# Autodesk Inventor assembly: staticFrame
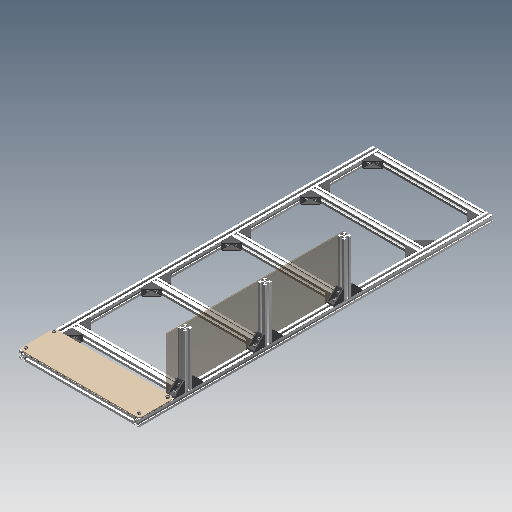
[picture p0: Inventor's stored thumbnail of the model, 512x512]
Saved by Autodesk Inventor 2018 (Build 220112000, 112)
## iProperties
Created: 2017-04-19
Part Number: staticFrame
Document SubType Name: Assembly
Designer: sawaiz
Author: sawaiz
## Documents named in this file (7)
- C:\Users\sawaiz\OneDrive\projects\sPhenixTileTestStand\frame\staticFrame.iam
- C:\Users\sawaiz\OneDrive\projects\sPhenixTileTestStand\frame\base.iam
- C:\Users\sawaiz\OneDrive\projects\sPhenixTileTestStand\frame\span.iam
- C:\Users\sawaiz\OneDrive\projects\sPhenixTileTestStand\frame\verticalStop.iam
- C:\Users\sawaiz\OneDrive\projects\sPhenixTileTestStand\frame\supportPlate.iam
- C:\Users\sawaiz\OneDrive\projects\sPhenixTileTestStand\frame\wallPlate.ipt
- C:\Users\sawaiz\OneDrive\projects\sPhenixTileTestStand\sPhenixTileTestStand.xlsx
## Components (10 placed, 5 different names)
1. base:1 [sub-assembly] — Mate:1, Flush:1, Mate:3, Flush:5, Mate:4, Flush:6, Flush:7
2. supportPlate:1 [sub-assembly] — Mate:4, Flush:6, Flush:7, Mate:7, Mate:8
3. wallPlate:1 — Mate:5, Mate:6, Mate:7
4. span:1 [sub-assembly] — Mate:1, Flush:1, Flush:8
5. span:2 [sub-assembly] — Mate:6
6. span:3 [sub-assembly]
7. span:4 [sub-assembly]
8. verticalStop:1 [sub-assembly] — Mate:3, Flush:5, Mate:5, Mate:8, Flush:8
9. verticalStop:2 [sub-assembly]
10. verticalStop:3 [sub-assembly]
## Component patterns: (4 elements, first: span:1), (3 elements, first: verticalStop:1)
## Relationships (12: Mate 7, Flush 5)
- Mate:1: base:1 ↔ span:1
- Flush:1: base:1 ↔ span:1
- Mate:3: base:1 ↔ verticalStop:1
- Flush:5: base:1 ↔ verticalStop:1
- Mate:4: base:1 ↔ supportPlate:1
- Flush:6: base:1 ↔ supportPlate:1
- Flush:7: base:1 ↔ supportPlate:1
- Mate:5: wallPlate:1 ↔ verticalStop:1
- Mate:6: wallPlate:1 ↔ span:2
- Mate:7: supportPlate:1 ↔ wallPlate:1
- Mate:8: supportPlate:1 ↔ verticalStop:1
- Flush:8: span:1 ↔ verticalStop:1
## Named parameters: width = 300 mm, depth = 1000 mm, height = 150 mm, suppourtPlateLength = 100 mm, acrylicThickness = 3.125 mm
